# Autodesk Inventor assembly: Kettenradzusammensetzung_links
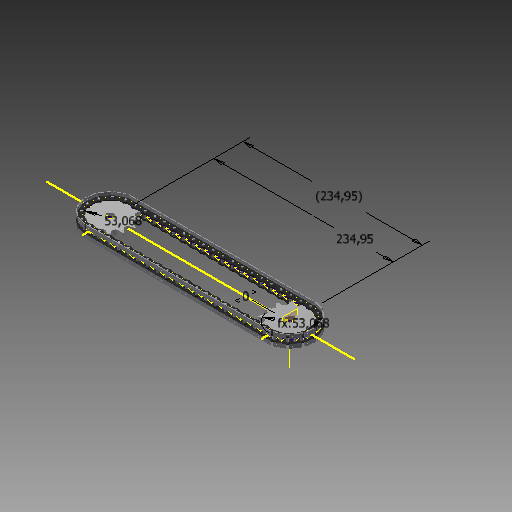
[picture p0: Inventor's stored thumbnail of the model, 512x512]
Saved by Autodesk Inventor 2018 (Build 220112000, 112)
## iProperties
Created: 2018-01-11
Part Number: Kettenradzusammensetzung_links
Material: Generisch
Document SubType Name: Assembly
Designer: Dominik
Author: Dominik
## Documents named in this file (4)
- C:\Users\Julian\Desktop\Schule\5AHME\Diplomarbeit\Git\fuettr_prototype\Mechanical\Inventorskizzen\Kettenradzusammensetzung_links.iam
- C:\Users\Julian\Desktop\Schule\5AHME\Diplomarbeit\Git\fuettr_prototype\Mechanical\Inventorskizzen\Kettenvorlage.ipt
- C:\Users\Julian\Desktop\Schule\5AHME\Diplomarbeit\Git\fuettr_prototype\Mechanical\Inventorskizzen\Kettenglied.ipt
- C:\Users\Julian\Desktop\Schule\5AHME\Diplomarbeit\Git\fuettr_prototype\Mechanical\Inventorskizzen\Kettenrad.ipt
## Components (53 placed, 3 different names)
1. Kettenvorlage:1 — Fluchtend:1, Fluchtend:2, Fluchtend:3, Passend:1, Passend:3, Drive, Passend:7
2. Roller Chain Sprocket1:1 — Passend:5, Winkel:2, Passend:6
3. Roller Chain Sprocket1:2 — Passend:8, Passend:9, Winkel:4
4. Kettenglied:1 — Passend:1, Winkel:1, Passend:2
5. Kettenglied:2
6. Kettenglied:3
7. Kettenglied:4
8. Kettenglied:5
9. Kettenglied:6
10. Kettenglied:7
11. Kettenglied:8
12. Kettenglied:9
13. Kettenglied:10
14. Kettenglied:11
15. Kettenglied:12
16. Kettenglied:13
17. Kettenglied:14
18. Kettenglied:15
19. Kettenglied:16
20. Kettenglied:17
21. Kettenglied:18
22. Kettenglied:19
23. Kettenglied:20
24. Kettenglied:21
25. Kettenglied:22
26. Kettenglied:23
27. Kettenglied:24
28. Kettenglied:25
29. Kettenglied:26
30. Kettenglied:27
31. Kettenglied:28
32. Kettenglied:29
33. Kettenglied:30
34. Kettenglied:31
35. Kettenglied:32
36. Kettenglied:33
37. Kettenglied:34
38. Kettenglied:35
39. Kettenglied:36
40. Kettenglied:37
41. Kettenglied:38
42. Kettenglied:39
43. Kettenglied:40
44. Kettenglied:41
45. Kettenglied:42
46. Kettenglied:43
47. Kettenglied:44
48. Kettenglied:45
49. Kettenglied:46
50. Kettenglied:47
51. Kettenglied:48
52. Kettenglied:49
53. Kettenglied:50
## Component patterns: (50 elements, first: Kettenglied:1)
## Relationships (16: Mate 9, Angle 4, Flush 3)
- Fluchtend:1 [Flush]: Kettenvorlage:1
- Fluchtend:2 [Flush]: Kettenvorlage:1
- Fluchtend:3 [Flush]: Kettenvorlage:1
- Passend:1 [Mate]: Kettenvorlage:1 ↔ Kettenglied:1
- Winkel:1 [Angle] (0 deg): Kettenglied:1
- Passend:2 [Mate]: Kettenglied:1
- Passend:3 [Mate] (234.95 mm): Kettenvorlage:1
- Drive [Mate] (234.95 mm): Kettenvorlage:1
- Passend:5 [Mate]: Roller Chain Sprocket1:1
- Winkel:2 [Angle] (0 deg): Roller Chain Sprocket1:1
- Passend:6 [Mate]: Roller Chain Sprocket1:1
- Passend:7 [Mate]: Kettenvorlage:1
- Winkel:3 [Angle] (0 deg)
- Passend:8 [Mate]: Roller Chain Sprocket1:2
- Passend:9 [Mate]: Roller Chain Sprocket1:2
- Winkel:4 [Angle] (180 deg): Roller Chain Sprocket1:2
